# Autodesk Inventor assembly: ballAndSocket
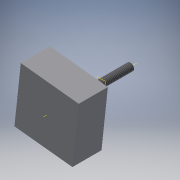
[picture p0: Inventor's stored thumbnail of the model, 180x180]
Saved by Autodesk Inventor 2019 (Build 230136000, 136)
## iProperties
Created: 2018-07-14
Part Number: ballAndSocket
Document SubType Name: Assembly
Designer: steele
Author: steele
## Documents named in this file (4)
- C:\git\CAD-Development\robSteele\HouseProjects\TableSaw\ballAndSocket.iam
- C:\git\CAD-Development\robSteele\HouseProjects\TableSaw\screwForAngledPiece.ipt
- C:\git\CAD-Development\robSteele\HouseProjects\TableSaw\ball.ipt
- C:\git\CAD-Development\robSteele\HouseProjects\TableSaw\socket.ipt
## Components (3 placed, 3 different names)
1. screwForAngledPiece:1 — Mate:1, Mate:2, Mate:3
2. ball:1 — Mate:1, Mate:2, Flush:1
3. socket:1 — Flush:1, Mate:3
## Relationships (4: Mate 3, Flush 1)
- Mate:1: screwForAngledPiece:1 ↔ ball:1
- Mate:2 (25.4 mm): screwForAngledPiece:1 ↔ ball:1
- Flush:1: ball:1 ↔ socket:1
- Mate:3: screwForAngledPiece:1 ↔ socket:1
## Named parameters: centerOfScrewToCenterOfBall = 25.4 mm
